# Autodesk Inventor assembly: Kostka
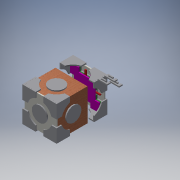
[picture p0: Inventor's stored thumbnail of the model, 180x180]
Saved by Autodesk Inventor 2018 (Build 220112000, 112)
## iProperties
Created: 2018-10-22
Part Number: Kostka
Material: Ogólny
Document SubType Name: Assembly
Designer: EWA
Author: EWA
## Documents named in this file (6)
- C:\Users\EWA\Documents\Inventor\Kostka\Kostka.iam
- C:\Users\EWA\Documents\Inventor\Kostka\Puszka.iam
- C:\Users\EWA\Documents\Inventor\Kostka\Naroznik.iam
- C:\Users\EWA\Documents\Inventor\Kostka\Mechanizm.iam
- C:\Users\EWA\Documents\Inventor\Kostka\Uchwyt_80.ipt
- C:\Users\EWA\Documents\Inventor\Kostka\Zamkek_puszka.ipt
## Components (19 placed, 5 different names)
1. Puszka:1 [sub-assembly] — Zestawiający:1, Zestawiający:2, Zestawiający:3, Zestawiający:4, Zestawiający:5, Zestawiający:6, Zestawiający:7, Zestawiający:8, Zestawiający:9, Zestawiający:10, Zestawiający:11, Zestawiający:12, Zestawiający:13, Sztywne:1, Sztywne:2, Sztywne:3, Sztywne:4, Sztywne:5, Zestawiający:26, Równoległy:3
2. Naroznik:1 [sub-assembly] — Zestawiający:6, Zestawiający:8, Zestawiający:12, Zestawiający:13
3. Naroznik:2 [sub-assembly] — Zestawiający:3, Zestawiający:4, Zestawiający:9
4. Naroznik:3 [sub-assembly] — Zestawiający:1, Zestawiający:7, Zestawiający:11, Równoległy:1, Równoległy:2
5. Naroznik:4 [sub-assembly] — Zestawiający:2, Zestawiający:5, Zestawiający:10
6. Uchwyt_80:1 — Sztywne:1
7. Mechanizm:1 [sub-assembly] — Zestawiający:14, Zestawiający:15, Zestawiający:16, Zestawiający:17, Zestawiający:18, Zestawiający:19, Zestawiający:20, Zestawiający:21, Zestawiający:22, Zestawiający:23, Zestawiający:24, Zestawiający:25
8. Naroznik:5 [sub-assembly] — Zestawiający:14, Zestawiający:15, Zestawiający:16
9. Naroznik:6 [sub-assembly] — Zestawiający:17, Zestawiający:18, Zestawiający:19, Równoległy:1, Równoległy:2
10. Naroznik:7 [sub-assembly] — Zestawiający:20, Zestawiający:21, Zestawiający:22
11. Naroznik:8 [sub-assembly] — Zestawiający:23, Zestawiający:24, Zestawiający:25
12. Uchwyt_80:2 — Sztywne:2
13. Uchwyt_80:3 — Sztywne:3
14. Uchwyt_80:4 — Sztywne:5
15. Uchwyt_80:6 — Sztywne:4
16. Zamkek_puszka:1 — Zestawiający:26, Równoległy:3
17. Zamkek_puszka:2
18. Zamkek_puszka:3
19. Zamkek_puszka:4
## Relationships (34: Mate 26, WeldJoint 5, Flush 3)
- Zestawiający:1 [Mate]: Puszka:1 ↔ Naroznik:3
- Zestawiający:2 [Mate]: Puszka:1 ↔ Naroznik:4
- Zestawiający:3 [Mate]: Puszka:1 ↔ Naroznik:2
- Zestawiający:4 [Mate]: Puszka:1 ↔ Naroznik:2
- Zestawiający:5 [Mate]: Puszka:1 ↔ Naroznik:4
- Zestawiający:6 [Mate]: Puszka:1 ↔ Naroznik:1
- Zestawiający:7 [Mate]: Puszka:1 ↔ Naroznik:3
- Zestawiający:8 [Mate]: Puszka:1 ↔ Naroznik:1
- Zestawiający:9 [Mate]: Puszka:1 ↔ Naroznik:2
- Zestawiający:10 [Mate]: Puszka:1 ↔ Naroznik:4
- Zestawiający:11 [Mate]: Puszka:1 ↔ Naroznik:3
- Zestawiający:12 [Mate]: Puszka:1 ↔ Naroznik:1
- Zestawiający:13 [Mate]: Puszka:1 ↔ Naroznik:1
- Sztywne:1 [WeldJoint]: Puszka:1 ↔ Uchwyt_80:1
- Zestawiający:14 [Mate]: Mechanizm:1 ↔ Naroznik:5
- Zestawiający:15 [Mate]: Mechanizm:1 ↔ Naroznik:5
- Zestawiający:16 [Mate]: Mechanizm:1 ↔ Naroznik:5
- Zestawiający:17 [Mate]: Mechanizm:1 ↔ Naroznik:6
- Zestawiający:18 [Mate]: Mechanizm:1 ↔ Naroznik:6
- Zestawiający:19 [Mate]: Mechanizm:1 ↔ Naroznik:6
- Zestawiający:20 [Mate]: Mechanizm:1 ↔ Naroznik:7
- Zestawiający:21 [Mate]: Mechanizm:1 ↔ Naroznik:7
- Zestawiający:22 [Mate]: Mechanizm:1 ↔ Naroznik:7
- Zestawiający:23 [Mate]: Mechanizm:1 ↔ Naroznik:8
- Zestawiający:24 [Mate]: Mechanizm:1 ↔ Naroznik:8
- Zestawiający:25 [Mate]: Mechanizm:1 ↔ Naroznik:8
- Sztywne:2 [WeldJoint]: Puszka:1 ↔ Uchwyt_80:2
- Sztywne:3 [WeldJoint]: Puszka:1 ↔ Uchwyt_80:3
- Sztywne:4 [WeldJoint]: Puszka:1 ↔ Uchwyt_80:6
- Sztywne:5 [WeldJoint]: Puszka:1 ↔ Uchwyt_80:4
- Równoległy:1 [Flush]: Naroznik:3 ↔ Naroznik:6
- Równoległy:2 [Flush]: Naroznik:3 ↔ Naroznik:6
- Zestawiający:26 [Mate]: Puszka:1 ↔ Zamkek_puszka:1
- Równoległy:3 [Flush]: Puszka:1 ↔ Zamkek_puszka:1
